# Autodesk Inventor assembly: 揺動節+ヘッケン_MIR
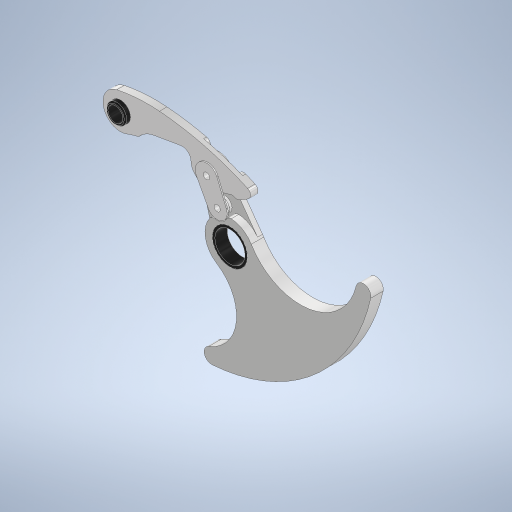
[picture p0: Inventor's stored thumbnail of the model, 512x512]
Saved by Autodesk Inventor 2023 (Build 270158000, 158)
## iProperties
Created: 2022-01-08
Part Number: 揺動節+ヘッケン_MIR
Document SubType Name: Assembly
Designer: acps
Author: acps
## Documents named in this file (7)
- C:\Users\muzho\Documents\srdc\srdc_2\脚\揺動節+ヘッケン_MIR.iam
- C:\Users\muzho\Documents\srdc\srdc_2\脚\揺動節_MIR.ipt
- C:\Users\muzho\Documents\srdc\srdc_2\脚\ヘッケン_MIR.ipt
- C:\Users\muzho\Documents\srdc\srdc_2\脚\ヘッケン抑え_MIR.ipt
- C:\Users\muzho\Documents\srdc\srdc_2\オイレス\w5f12-14n_MIR.ipt
- C:\Users\muzho\Documents\srdc\srdc_2\オイレス\w1.5f5-7n_MIR.ipt
- C:\Users\muzho\Documents\srdc\srdc_2\オイレス\w5f6-12a_MIR.ipt
## Components (6 placed, 6 different names)
1. 揺動節_MIR:1 — Insert:6, Insert:5
2. ヘッケン_MIR:1 — Insert:6, Insert:8, Mate:2, Mate:1, Insert:9, Insert:7
3. ヘッケン抑え_MIR:1 — Insert:8, Mate:2, Mate:1
4. w5f12-14n_MIR:1 — Insert:9
5. w1.5f5-7n_MIR:1 — Insert:7
6. w5f6-12a_MIR:1 — Insert:5
## Relationships (7: Insert 5, Mate 2)
- Insert:6: 揺動節_MIR:1 ↔ ヘッケン_MIR:1
- Insert:8: ヘッケン_MIR:1 ↔ ヘッケン抑え_MIR:1
- Mate:2: ヘッケン_MIR:1 ↔ ヘッケン抑え_MIR:1
- Mate:1: ヘッケン_MIR:1 ↔ ヘッケン抑え_MIR:1
- Insert:9: ヘッケン_MIR:1 ↔ w5f12-14n_MIR:1
- Insert:7: ヘッケン_MIR:1 ↔ w1.5f5-7n_MIR:1
- Insert:5: 揺動節_MIR:1 ↔ w5f6-12a_MIR:1
